# Autodesk Inventor assembly: flapper
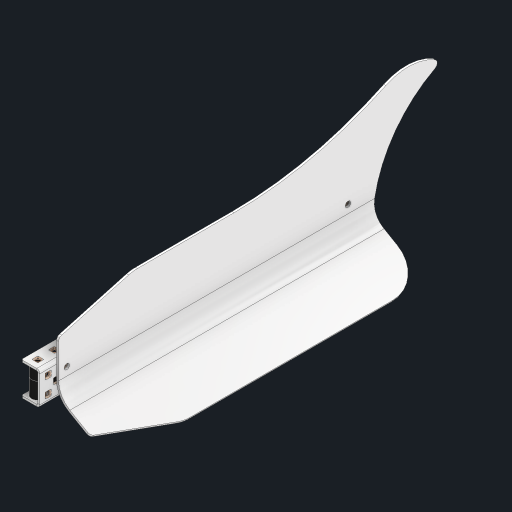
[picture p0: Inventor's stored thumbnail of the model, 512x512]
Saved by Autodesk Inventor 2024 (Build 280153000, 153)
## iProperties
Created: 2023-08-17
Part Number: flapper
Document SubType Name: Assembly
Designer: avere
Author: avere
## Documents named in this file (6)
- D:\cad\scrap_v0.1\chassis\flapper.iam
- D:\cad\VEX-CAD-Inventor-1.41\Structure\C Channel\Aluminum 1x2x1\Alu C 1x2x1x20.ipt
- D:\cad\VEX-CAD-Inventor-1.41\Motion\Spacers\Spacer Nylon .375 OD\NSpacer .375 OD x .375.ipt
- D:\vex_robotics\hardware\cad\VEX-CAD-Inventor-1.41\Motion\Spacers\Spacer Nylon .375 OD.ipt
- D:\cad\VEX-CAD-Inventor-1.41\Motion\Spacers\Spacer Nylon .375 OD\NSpacer .375 OD x .500.ipt
- D:\cad\scrap_v0.1\chassis\custom_parts\wedge.ipt
## Components (4 placed, 4 different names)
1. Alu C 1x2x1x20:1 — Insert:2, Insert:3, Mate:1
2. NSpacer .375 OD x .375:1 — Insert:1
3. NSpacer .375 OD x .500:2 — Insert:1, Insert:2
4. wedge:1 — Insert:3, Mate:1
## Relationships (4: Insert 3, Mate 1)
- Insert:1: NSpacer .375 OD x .375:1 ↔ NSpacer .375 OD x .500:2
- Insert:2: Alu C 1x2x1x20:1 ↔ NSpacer .375 OD x .500:2
- Insert:3: Alu C 1x2x1x20:1 ↔ wedge:1
- Mate:1: Alu C 1x2x1x20:1 ↔ wedge:1
